# Autodesk Inventor assembly: foot
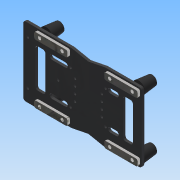
[picture p0: Inventor's stored thumbnail of the model, 180x180]
Saved by Autodesk Inventor 2015 (Build 190159000, 159)
## iProperties
Created: 2017-02-14
Part Number: foot
Document SubType Name: Assembly
Designer: Gregwar
Author: Gregwar
## Documents named in this file (5)
- C:\Users\Gregwar\Desktop\Design\foot\foot.iam
- C:\Users\Gregwar\Desktop\Design\foot\foot.ipt
- C:\Users\Gregwar\Desktop\Design\foot\cell.ipt
- C:\Users\Gregwar\Desktop\Design\foot\nylon_spacer.ipt
- C:\Users\Gregwar\Desktop\Design\foot\cleat.ipt
## Components (13 placed, 4 different names)
1. foot:1 — Placage:1, Placage:2, Placage:3, Placage:5, Placage:12, Placage:13, Placage:14, Placage:23, Placage:24, Placage:25, Placage:26, Placage:27, Placage:28
2. cell:1 — Placage:1, Placage:2, Placage:3, Placage:4, Placage:7
3. nylon_spacer:1 — Placage:4, Placage:5, Placage:6
4. cleat:1 — Placage:6, Placage:7
5. cell:2 — Placage:11, Placage:12, Placage:13, Placage:14
6. nylon_spacer:2 — Placage:11
7. cleat:2
8. cell:3 — Placage:24, Placage:25, Placage:28
9. nylon_spacer:3
10. cleat:3
11. cell:4 — Placage:23, Placage:26, Placage:27
12. nylon_spacer:4
13. cleat:4
## Relationships (28: Mate 28)
- Placage:1 [Mate]: foot:1 ↔ cell:1
- Placage:2 [Mate]: foot:1 ↔ cell:1
- Placage:3 [Mate]: foot:1 ↔ cell:1
- Placage:4 [Mate]: cell:1 ↔ nylon_spacer:1
- Placage:5 [Mate]: foot:1 ↔ nylon_spacer:1
- Placage:6 [Mate]: nylon_spacer:1 ↔ cleat:1
- Placage:7 [Mate]: cell:1 ↔ cleat:1
- [Mate]: cell:2 ↔ nylon_spacer:2
- [Mate]: nylon_spacer:2 ↔ cleat:2
- [Mate]: cell:2 ↔ cleat:2
- Placage:11 [Mate]: cell:2 ↔ nylon_spacer:2
- Placage:12 [Mate]: foot:1 ↔ cell:2
- Placage:13 [Mate]: foot:1 ↔ cell:2
- Placage:14 [Mate]: foot:1 ↔ cell:2
- [Mate]: cell:3 ↔ nylon_spacer:3
- [Mate]: nylon_spacer:3 ↔ cleat:3
- [Mate]: cell:3 ↔ cleat:3
- [Mate]: cell:3 ↔ nylon_spacer:3
- [Mate]: cell:4 ↔ nylon_spacer:4
- [Mate]: nylon_spacer:4 ↔ cleat:4
- [Mate]: cell:4 ↔ cleat:4
- [Mate]: cell:4 ↔ nylon_spacer:4
- Placage:23 [Mate]: foot:1 ↔ cell:4
- Placage:24 [Mate]: foot:1 ↔ cell:3
- Placage:25 [Mate]: foot:1 ↔ cell:3
- Placage:26 [Mate]: foot:1 ↔ cell:4
- Placage:27 [Mate]: foot:1 ↔ cell:4
- Placage:28 [Mate]: foot:1 ↔ cell:3
## Named parameters: d7_d3 = 0 mm, d8_d5 = 0 mm, d9_d6 = 0 mm, d14_d7_d3 = 0 mm, d15_d8_d5 = 0 mm, d16_d9_d6 = 0 mm, d17_d10 = 0 mm, d18_d7_d3 = 0 mm, d19_d8_d5 = 0 mm, d20_d9_d6 = 0 mm, d21_d10 = 0 mm
